# Autodesk Inventor assembly: Big table
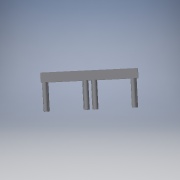
[picture p0: Inventor's stored thumbnail of the model, 180x180]
Saved by Autodesk Inventor 2019 (Build 230136000, 136)
## iProperties
Created: 2018-12-11
Part Number: Big table
Document SubType Name: Assembly
Designer: User
Author: User
## Documents named in this file (2)
- C:\Robotics\CAD\2018-19_CAD\will\Big table.iam
- C:\Robotics\CAD\2018-19_CAD\will\Table.ipt
## Components (4 placed, 1 different names)
1. Table:1 — Flush:1, Flush:2, Mate:1, Flush:3, Flush:4, Mate:2
2. Table:2 — Flush:1, Flush:2, Mate:1
3. Table:4 — Flush:3, Flush:4, Mate:2, Flush:5, Mate:3, Flush:6
4. Table:5 — Flush:5, Mate:3, Flush:6
## Relationships (9: Flush 6, Mate 3)
- Flush:1: Table:1 ↔ Table:2
- Flush:2: Table:1 ↔ Table:2
- Mate:1: Table:1 ↔ Table:2
- Flush:3: Table:1 ↔ Table:4
- Flush:4: Table:1 ↔ Table:4
- Mate:2: Table:1 ↔ Table:4
- Flush:5: Table:4 ↔ Table:5
- Mate:3: Table:4 ↔ Table:5
- Flush:6: Table:4 ↔ Table:5
